# Autodesk Inventor assembly: Footrest
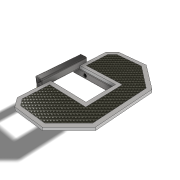
[picture p0: Inventor's stored thumbnail of the model, 180x180]
Saved by Autodesk Inventor 2020 (Build 240168000, 168)
## iProperties
Created: 2019-05-20
Part Number: Footrest
Document SubType Name: Assembly
Designer: chitl
Mass: 425.05 g
Surface Area: 530.728 cm^2
Volume: 123.385 cm^3
Density: 3.4449 g/cm^3
Author: chitl
## Documents named in this file (5)
- C:\Users\chitl\Desktop\OneWheel\Wheel Assembled\Pedal\Footrest\Footrest.iam
- C:\Users\chitl\Desktop\OneWheel\Wheel Assembled\Pedal\Footrest\Footrest_Aluminum_Top.ipt
- C:\Users\chitl\Desktop\OneWheel\Wheel Assembled\Pedal\Footrest\Footrest_Steel_Frame_0.5\Frame\Frame 1558256322523.iam
- C:\Users\chitl\Desktop\OneWheel\Wheel Assembled\Handle\Footrest_v2.ipt
- C:\Users\chitl\Desktop\OneWheel\Wheel Assembled\Pedal\Footrest\grip_tape.ipt
## Components (4 placed, 4 different names)
1. Frame 1558256322523:1 [sub-assembly] — Mate:1, Mate:2, Mate:3, Mate:4
2. Footrest_Aluminum_Top:1 — Mate:1, Mate:2
3. Footrest_v2:1 — Mate:3, Mate:4, Mate:5
4. grip_tape:1 — Mate:5
## Relationships (5: Mate 5)
- Mate:1: Frame 1558256322523:1 ↔ Footrest_Aluminum_Top:1
- Mate:2: Frame 1558256322523:1 ↔ Footrest_Aluminum_Top:1
- Mate:3: Frame 1558256322523:1 ↔ Footrest_v2:1
- Mate:4: Frame 1558256322523:1 ↔ Footrest_v2:1
- Mate:5: Footrest_v2:1 ↔ grip_tape:1
